# Autodesk Inventor assembly: M2-ヘッケンv2
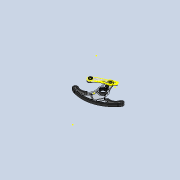
[picture p0: Inventor's stored thumbnail of the model, 180x180]
Saved by Autodesk Inventor 2020 (Build 240168000, 168)
## iProperties
Created: 2020-10-27
Part Number: M2-ヘッケンv2
Document SubType Name: Assembly
Designer: AA19065
Mass: 11.1235 g
Surface Area: 107.349 cm^2
Volume: 7.82402 cm^3
Density: 1.42171 g/cm^3
Author: AA19065
## Documents named in this file (9)
- C:\Users\happy\OneDrive\ドキュメント\賢一ファイル\SRDC\試作10-2\アセンブリ\M2-ヘッケンv2.iam
- C:\Users\happy\OneDrive\ドキュメント\賢一ファイル\SRDC\試作10-2\脚クランク\M2-揺動節.ipt
- C:\Users\happy\OneDrive\ドキュメント\賢一ファイル\SRDC\試作10-2\脚クランク\M2-揺動節抑え.ipt
- C:\Users\happy\OneDrive\ドキュメント\賢一ファイル\SRDC\試作10-2\軸受け\M2-オイレスw1.5f5-7n.ipt
- C:\Users\happy\OneDrive\ドキュメント\賢一ファイル\SRDC\試作10-2\軸受け\M2-オイレスw5f6-10a.ipt
- C:\Users\happy\OneDrive\ドキュメント\賢一ファイル\SRDC\試作10-2\軸受け\M2-オイレスw5f12-14n.ipt
- C:\Users\happy\OneDrive\ドキュメント\賢一ファイル\SRDC\試作10-2\ヘッケン\M2-ヘッケンv2.ipt
- C:\Users\happy\OneDrive\ドキュメント\賢一ファイル\SRDC\試作10-2\ヘッケン\M2-脚ゴム.ipt
- C:\Users\happy\OneDrive\ドキュメント\賢一ファイル\SRDC\試作10-2\ねじ\M2-m3皿ネジ5 (1).ipt
## Components (9 placed, 8 different names)
1. M2-揺動節:1 — 挿入:17, 挿入:8
2. M2-揺動節抑え:1 — 挿入:13, 挿入:12
3. M2-オイレスw1.5f5-7n:1 — 挿入:17, 挿入:10
4. M2-オイレスw5f6-10a:1 — 挿入:8
5. M2-オイレスw5f12-14n:1 — 挿入:11
6. M2-ヘッケンv2:1 — 挿入:13, 挿入:12, 挿入:11, 挿入:10, メイト:1, 挿入:16, 挿入:19, 挿入:18
7. M2-脚ゴム:1 — メイト:1, 挿入:16
8. M2-m3皿ネジ5 (1):1 — 挿入:19
9. M2-m3皿ネジ5 (1):2 — 挿入:18
## Relationships (10: Insert 9, Mate 1)
- 挿入:17 [Insert]: M2-揺動節:1 ↔ M2-オイレスw1.5f5-7n:1
- 挿入:8 [Insert]: M2-揺動節:1 ↔ M2-オイレスw5f6-10a:1
- 挿入:13 [Insert]: M2-揺動節抑え:1 ↔ M2-ヘッケンv2:1
- 挿入:12 [Insert]: M2-揺動節抑え:1 ↔ M2-ヘッケンv2:1
- 挿入:11 [Insert]: M2-オイレスw5f12-14n:1 ↔ M2-ヘッケンv2:1
- 挿入:10 [Insert]: M2-オイレスw1.5f5-7n:1 ↔ M2-ヘッケンv2:1
- メイト:1 [Mate] (-1.34 mm): M2-ヘッケンv2:1 ↔ M2-脚ゴム:1
- 挿入:16 [Insert]: M2-ヘッケンv2:1 ↔ M2-脚ゴム:1
- 挿入:19 [Insert]: M2-ヘッケンv2:1 ↔ M2-m3皿ネジ5 (1):1
- 挿入:18 [Insert]: M2-ヘッケンv2:1 ↔ M2-m3皿ネジ5 (1):2
